# Autodesk Inventor assembly: SolarGearRingWithBlind
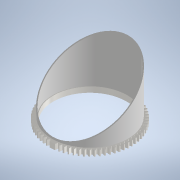
[picture p0: Inventor's stored thumbnail of the model, 180x180]
Saved by Autodesk Inventor 2021 (Build 250183000, 183)
## iProperties
Created: 2021-03-13
Part Number: SolarGearRingWithBlind
Document SubType Name: Assembly
Designer: allen
Author: allen
## Documents named in this file (3)
- C:\Users\allen\Downloads\repos\YingXao\YingXao_Mechanical\In Development\SolarGearRingWithBlind.iam
- C:\Users\allen\Downloads\repos\YingXao\YingXao_Mechanical\In Development\SolarGear_v5\Design Accelerator\Spur Gear21.ipt
- C:\Users\allen\Downloads\repos\YingXao\YingXao_Mechanical\In Development\SolarPanel.ipt
## Components (2 placed, 2 different names)
1. Spur Gear2:1 — Mate:1, Mate:2
2. SolarPanel:1 — Mate:1, Mate:2
## Relationships (2: Mate 2)
- Mate:1: Spur Gear2:1 ↔ SolarPanel:1
- Mate:2: Spur Gear2:1 ↔ SolarPanel:1
